# Autodesk Inventor assembly: VersaWheel Configurator
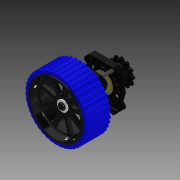
[picture p0: Inventor's stored thumbnail of the model, 180x180]
Saved by Autodesk Inventor 2022 (Build 260153000, 153)
## iProperties
Created: 2021-12-11
Part Number: VersaWheel Configurator
Document SubType Name: Assembly
Designer: Max Boord
Author: Max Boord
## iProperties of the stored document MemberDocs/xKavof0oyKcrsz2a5Zln5g1o0Ze
Created: 2021-12-11
Part Number: VersaWheel Configurator
Document SubType Name: Assembly
Mass: 595.394 g
Surface Area: 1093.39 cm^2
Volume: 176.36 cm^3
Density: 3.37601 g/cm^3
## iProperties of the stored document MemberDocs/xCuhoath5H0oh0c4sRnknl0ad1f
Created: 2021-12-11
Part Number: VersaWheel Configurator
Document SubType Name: Assembly
Mass: 595.394 g
Surface Area: 1093.39 cm^2
Volume: 176.36 cm^3
Density: 3.37601 g/cm^3
## iProperties of the stored document MemberDocs/x11aqephyIc3nsah0Sedduv5mFh
Created: 2021-12-11
Part Number: VersaWheel Configurator
Document SubType Name: Assembly
Mass: 595.394 g
Surface Area: 1093.39 cm^2
Volume: 176.36 cm^3
Density: 3.37601 g/cm^3
## iProperties of the stored document MemberDocs/xJkytpkcnEsn5gh20DplldbomNd
Created: 2021-12-11
Part Number: VersaWheel Configurator
Document SubType Name: Assembly
Mass: 595.394 g
Surface Area: 1093.39 cm^2
Volume: 176.36 cm^3
Density: 3.37601 g/cm^3
## iProperties of the stored document MemberDocs/xPda1jvqgM0n25ka0KrmnxploXd
Created: 2021-12-11
Part Number: VersaWheel Configurator
Document SubType Name: Assembly
Mass: 595.394 g
Surface Area: 1093.39 cm^2
Volume: 176.36 cm^3
Density: 3.37601 g/cm^3
## iProperties of the stored document MemberDocs/xOycl5yj1Mkam4njnN1axot5lNc
Created: 2021-12-11
Part Number: VersaWheel Configurator
Document SubType Name: Assembly
Mass: 595.394 g
Surface Area: 1093.39 cm^2
Volume: 176.36 cm^3
Density: 3.37601 g/cm^3
## iProperties of the stored document MemberDocs/xTmgljwieNkiy1fcf15cxnqeoYc
Created: 2021-12-11
Part Number: VersaWheel Configurator
Document SubType Name: Assembly
Mass: 595.394 g
Surface Area: 1093.39 cm^2
Volume: 176.36 cm^3
Density: 3.37601 g/cm^3
## iProperties of the stored document MemberDocs/xVde5yltuAso2rnbgL5gfk11iAe
Created: 2021-12-11
Part Number: VersaWheel Configurator
Document SubType Name: Assembly
## Documents named in this file (56)
- C:\Users\Cal\Desktop\Robotics\Design\Collaborative\Collaborative Parts Library\Drivetrains\Wheel Configurations\VersaWheel Configurator.iam
- C:\Users\Max Boord\Downloads\217-3437.ipt
- E:\Middleton Robotics\Collaborative Robots\Collaborative Part Library\Power Transfer\Bearing Blocks\VersaBlock V2 (217-6111).ipt
- E:\Middleton Robotics\Collaborative Robots\Collaborative Part Library\Power Transfer\Bearings\FR8 Hex.ipt
- E:\Middleton Robotics\Collaborative Robots\Collaborative Part Library\Power Transfer\Bearings.ipt
- E:\Middleton Robotics\Collaborative Robots\Collaborative Part Library\Power Transfer\VexPro Sprockets.ipt
- E:\Middleton Robotics\Collaborative Robots\Collaborative Part Library\Power Transfer\Sprockets\VexPro 12T 35 Chain 500 Hex Bore Double Sprocket (Steel).ipt
- E:\Middleton Robotics\Collaborative Robots\Collaborative Part Library\Hardware\Spacers & Standoffs.ipt
- E:\Middleton Robotics\Collaborative Robots\Collaborative Part Library\Shaft Retention\Snaprings\Snapring for 0.5in Shaft (0.461in).ipt
- E:\Middleton Robotics\Collaborative Robots\Collaborative Part Library\Shaft Retention\Snaprings.ipt
- E:\Middleton Robotics\Collaborative Robots\Collaborative Part Library\Hardware\Spacers & Standoffs\VexPro 500 Hex Spacer 0.125in.ipt
- E:\Middleton Robotics\Collaborative Robots\Collaborative Part Library\Wheels and Rollers\Wheels\WCP AL Wheel 4 x 1.5 (WCP-0075) With tread.iam
- E:\Middleton Robotics\Collaborative Robots\Collaborative Part Library\Wheels and Rollers\Wheels\VexPro 6x2 Pneumatic Wheel.ipt
- E:\Middleton Robotics\Collaborative Robots\Collaborative Part Library\Hardware\Washers\Washer 0.265ID 0.688OD 0.055Thick.ipt
- E:\Middleton Robotics\Collaborative Robots\Collaborative Part Library\Hardware\Washers.ipt
- E:\Middleton Robotics\Collaborative Robots\Collaborative Part Library\Hardware\Machine Screws\1(_FS)4-20 UNCx0.5 Button Head Cap Screw.ipt
- E:\Middleton Robotics\Collaborative Robots\Collaborative Part Library\Hardware\Machine Screws.ipt
- E:\Middleton Robotics\Collaborative Robots\Collaborative Part Library\Hardware\Machine Screws\10-32 UNFx1.5 Socket Head Cap Screw.ipt
- E:\Middleton Robotics\Collaborative Robots\Collaborative Part Library\Wheels and Rollers\Wheels\Omni 4 x 2 (VexPro 217-2584).ipt
- E:\Middleton Robotics\Collaborative Robots\Collaborative Part Library\Power Transfer\Hubs\VersaHub .500 Hex (Plastic).ipt
- E:\Middleton Robotics\Collaborative Robots\Collaborative Part Library\Power Transfer\Hubs\VersaHub .500 Hex.ipt
- E:\Middleton Robotics\Collaborative Robots\Collaborative Part Library\Hardware\Machine Screws\8-32 UNCx0.5 Button Head Cap Screw.ipt
- E:\Exploding Bacon\Parts Library\Wheels\WCP 8 Inch Pneumatic Wheel (WCP-0049).ipt
- C:\Users\Cal\Desktop\Robotics\Design\Collaborative\Collaborative Parts Library\Drivetrains\VersaChassis Parts\217-3437.ipt
- C:\Users\Cal\Desktop\Robotics\Design\Collaborative\Collaborative Parts Library\Power Transfer\Bearing Blocks\VersaBlock V2 (217-6111).ipt
- C:\Users\Cal\Desktop\Robotics\Design\Collaborative\Collaborative Parts Library\Power Transfer\Bearings and Bushings\Bearings\FR8 Hex.ipt
- C:\Users\Cal\Desktop\Robotics\Design\Collaborative\Collaborative Parts Library\Shaft Retention\Snaprings\Snapring for 0.5in Shaft (0.461in).ipt
- C:\Users\Cal\Desktop\Robotics\Design\Collaborative\Collaborative Parts Library\Hardware\Spacers\Spacers & Standoffs\VexPro 500 Hex Spacer 0.125in.ipt
- C:\Users\Cal\Desktop\Robotics\Design\Collaborative\Collaborative Parts Library\Wheels\Pneumatic Wheels\6 in x 2 in  Pneumatic Wheel.ipt
- C:\Users\Cal\Desktop\Robotics\Design\Collaborative\Collaborative Parts Library\Hardware\Fasteners\Washers\Washer 0.265ID 0.688OD 0.055Thick.ipt
- C:\Users\Cal\Desktop\Robotics\Design\Collaborative\Collaborative Parts Library\Hardware\Fasteners\Machine Screws\1(_FS)4-20 UNCx0.5 Button Head Cap Screw.ipt
- C:\Users\Cal\Desktop\Robotics\Design\Collaborative\Collaborative Parts Library\Hardware\Fasteners\Machine Screws\10-32 UNFx1.5 Socket Head Cap Screw.ipt
- C:\Users\Cal\Desktop\Robotics\Design\Collaborative\Collaborative Parts Library\Wheels\Omni Wheels\Omni 4 x 2 (VexPro 217-2584).ipt
- C:\Users\Cal\Desktop\Robotics\Design\Collaborative\Collaborative Parts Library\Power Transfer\Hubs (Hex and Key)\VersaHub .500 Hex (Plastic).ipt
- C:\Users\Cal\Desktop\Robotics\Design\Collaborative\Collaborative Parts Library\Power Transfer\Hubs (Hex and Key)\VersaHub .500 Hex.ipt
- C:\Users\Cal\Desktop\Robotics\Design\Collaborative\Collaborative Parts Library\Hardware\Fasteners\Machine Screws\8-32 UNCx0.5 Button Head Cap Screw.ipt
- E:\Middleton Robotics\Collaborative Robots\Collaborative Part Library\Wheels and Rollers\Wheels\WCP 8 Inch Pneumatic Wheel (WCP-0049).ipt
- C:\Users\Cal\Desktop\Robotics\Design\Collaborative\Collaborative Parts Library\Wheels\Hard Wheels\WCP Nitrile Wheel & Tread.ipt
- C:\Users\Cal\Desktop\Robotics\Design\Collaborative\Collaborative Parts Library\Power Transfer\Sprockets\Sprockets\VexPro 12T 35 Chain 500 Hex Bore Double Sprocket.ipt
- E:\Middleton Robotics\Collaborative Robots\Collaborative Part Library\Power Transfer\Sprockets\VexPro Sprockets.ipt
- E:\Middleton Robotics\Collaborative Robots\Collaborative Part Library\Drivetrains\VersaChassis Parts\217-3437.ipt
- E:\Middleton Robotics\Collaborative Robots\Collaborative Part Library\Power Transfer\Bearings and Bushings\Bearings\FR8 Hex.ipt
- E:\Middleton Robotics\Collaborative Robots\Collaborative Part Library\Hardware\Spacers\Spacers & Standoffs\VexPro 500 Hex Spacer 0.125in.ipt
- E:\Middleton Robotics\Collaborative Robots\Collaborative Part Library\Wheels\6 in x 2 in  Pneumatic Wheel.ipt
- E:\Middleton Robotics\Collaborative Robots\Collaborative Part Library\Hardware\Fasteners\Washers\Washer 0.265ID 0.688OD 0.055Thick.ipt
- E:\Middleton Robotics\Collaborative Robots\Collaborative Part Library\Hardware\Fasteners\Machine Screws\1(_FS)4-20 UNCx0.5 Button Head Cap Screw.ipt
- E:\Middleton Robotics\Collaborative Robots\Collaborative Part Library\Hardware\Fasteners\Machine Screws\10-32 UNFx1.5 Socket Head Cap Screw.ipt
- E:\Middleton Robotics\Collaborative Robots\Collaborative Part Library\Wheels\Omni 4 x 2 (VexPro 217-2584).ipt
- E:\Middleton Robotics\Collaborative Robots\Collaborative Part Library\Power Transfer\Hubs (Hex and Key)\VersaHub .500 Hex (Plastic).ipt
- E:\Middleton Robotics\Collaborative Robots\Collaborative Part Library\Power Transfer\Hubs (Hex and Key)\VersaHub .500 Hex.ipt
- E:\Middleton Robotics\Collaborative Robots\Collaborative Part Library\Hardware\Fasteners\Machine Screws\8-32 UNCx0.5 Button Head Cap Screw.ipt
- E:\Middleton Robotics\Collaborative Robots\Collaborative Part Library\Wheels\WCP Nitrile Wheel & Tread.ipt
- E:\Middleton Robotics\Collaborative Robots\Collaborative Part Library\Power Transfer\Sprockets\Sprockets\VexPro 12T 35 Chain 500 Hex Bore Double Sprocket.ipt
- C:\Users\Cal\Desktop\Robotics\Design\Collaborative\Collaborative Parts Library\Wheels\6 in x 2 in  Pneumatic Wheel.ipt
- C:\Users\Cal\Desktop\Robotics\Design\Collaborative\Collaborative Parts Library\Wheels\Omni 4 x 2 (VexPro 217-2584).ipt
- C:\Users\Cal\Desktop\Robotics\Design\Collaborative\Collaborative Parts Library\Wheels\WCP Nitrile Wheel & Tread.ipt
## Components (31 placed, 16 different names)
1. 217-3437:1 — Insert:6, Insert:7, Mate:2, Insert:10
2. VersaBlock V2 (217-6111):1 — Insert:1, Mate:1, Symmetry:1
3. FR8 Hex:1 — Insert:1, Insert:3, Insert:5
4. VexPro 12T 35 Chain 500 Hex Bore Double Sprocket (Steel):2 — Insert:4, Insert:6
5. VexPro 500 Hex Spacer 0.125in:2 — Insert:3, Insert:4
6. VersaBlock V2 (217-6111):2 — Mate:1, Symmetry:1, Mate:3, Insert:11, Insert:12
7. FR8 Hex:2 — Insert:5, Insert:8, Insert:17, Insert:18, Insert:19, Insert:20
8. Snapring for 0.5in Shaft (0.461in):1 — Insert:7
9. WCP AL Wheel 4 x 1.5 (WCP-0075) With tread:1 [sub-assembly] — Insert:8
10. 10-32 UNFx1.5 Socket Head Cap Screw:2 — Insert:12
11. 10-32 UNFx1.5 Socket Head Cap Screw:3 — Insert:11
12. VexPro 6x2 Pneumatic Wheel:1 — Insert:18
13. Washer 0.265ID 0.688OD 0.055Thick:1 — Insert:9, Insert:10
14. 1(_FS)4-20 UNCx0.5 Button Head Cap Screw:1 — Insert:9
15. Omni 4 x 2 (VexPro 217-2584):1 — Insert:13, Mate:4, Insert:14, Mate:5
16. VersaHub .500 Hex (Plastic):1 — Insert:14, Mate:5, Insert:15
17. VersaHub .500 Hex:1 — Insert:13, Mate:4, Insert:16, Insert:17
18. WCP 8 Inch Pneumatic Wheel (WCP-0049):1 — Insert:19
19. VexPro 500 Hex Spacer 0.125in:3 — Insert:20
20. 8-32 UNCx0.5 Button Head Cap Screw:4 — Insert:15
21. 8-32 UNCx0.5 Button Head Cap Screw:10 — Insert:16
22. 8-32 UNCx0.5 Button Head Cap Screw:5
23. 8-32 UNCx0.5 Button Head Cap Screw:11
24. 8-32 UNCx0.5 Button Head Cap Screw:6
25. 8-32 UNCx0.5 Button Head Cap Screw:12
26. 8-32 UNCx0.5 Button Head Cap Screw:7
27. 8-32 UNCx0.5 Button Head Cap Screw:13
28. 8-32 UNCx0.5 Button Head Cap Screw:8
29. 8-32 UNCx0.5 Button Head Cap Screw:14
30. 8-32 UNCx0.5 Button Head Cap Screw:9
31. 8-32 UNCx0.5 Button Head Cap Screw:15
## Component patterns: (6 elements, first: 8-32 UNCx0.5 Button Head Cap Screw:4 + 8-32 UNCx0.5 Button Head Cap Screw:10)
## Relationships (26: Insert 20, Mate 5, Symmetry 1)
- Insert:1: VersaBlock V2 (217-6111):1 ↔ FR8 Hex:1
- [Insert]: VersaBlock V2 (217-6111):2 ↔ FR8 Hex:2
- Insert:3: FR8 Hex:1 ↔ VexPro 500 Hex Spacer 0.125in:2
- Insert:4: VexPro 12T 35 Chain 500 Hex Bore Double Sprocket (Steel):2 ↔ VexPro 500 Hex Spacer 0.125in:2
- Insert:5 (25.4 mm): FR8 Hex:1 ↔ FR8 Hex:2
- Mate:1: VersaBlock V2 (217-6111):1 ↔ VersaBlock V2 (217-6111):2
- Insert:6: 217-3437:1 ↔ VexPro 12T 35 Chain 500 Hex Bore Double Sprocket (Steel):2
- Insert:7: 217-3437:1 ↔ Snapring for 0.5in Shaft (0.461in):1
- Symmetry:1: VersaBlock V2 (217-6111):1 ↔ VersaBlock V2 (217-6111):2
- Mate:2: 217-3437:1
- Mate:3: VersaBlock V2 (217-6111):2
- Insert:8: FR8 Hex:2 ↔ WCP AL Wheel 4 x 1.5 (WCP-0075) With tread:1
- Insert:9: Washer 0.265ID 0.688OD 0.055Thick:1 ↔ 1(_FS)4-20 UNCx0.5 Button Head Cap Screw:1
- Insert:10: 217-3437:1 ↔ Washer 0.265ID 0.688OD 0.055Thick:1
- Insert:11: VersaBlock V2 (217-6111):2 ↔ 10-32 UNFx1.5 Socket Head Cap Screw:3
- Insert:12: VersaBlock V2 (217-6111):2 ↔ 10-32 UNFx1.5 Socket Head Cap Screw:2
- Insert:13: Omni 4 x 2 (VexPro 217-2584):1 ↔ VersaHub .500 Hex:1
- Mate:4: Omni 4 x 2 (VexPro 217-2584):1 ↔ VersaHub .500 Hex:1
- Insert:14: Omni 4 x 2 (VexPro 217-2584):1 ↔ VersaHub .500 Hex (Plastic):1
- Mate:5: Omni 4 x 2 (VexPro 217-2584):1 ↔ VersaHub .500 Hex (Plastic):1
- Insert:15: VersaHub .500 Hex (Plastic):1 ↔ 8-32 UNCx0.5 Button Head Cap Screw:4
- Insert:16: VersaHub .500 Hex:1 ↔ 8-32 UNCx0.5 Button Head Cap Screw:10
- Insert:17 (3.175 mm): FR8 Hex:2 ↔ VersaHub .500 Hex:1
- Insert:18: FR8 Hex:2 ↔ VexPro 6x2 Pneumatic Wheel:1
- Insert:19: FR8 Hex:2 ↔ WCP 8 Inch Pneumatic Wheel (WCP-0049):1
- Insert:20: FR8 Hex:2 ↔ VexPro 500 Hex Spacer 0.125in:3
## Named parameters: d1_d0 = 0 mm
